# Autodesk Inventor assembly: tail
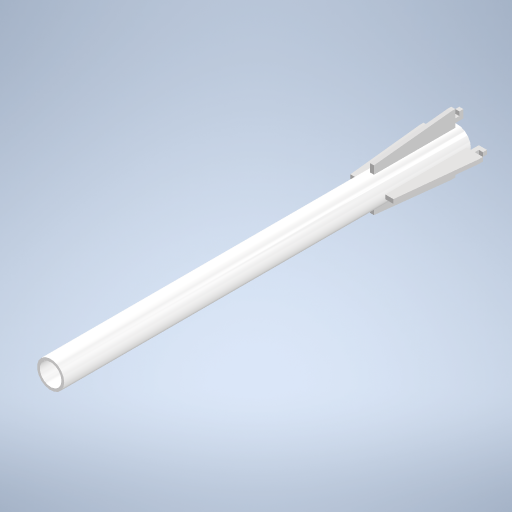
[picture p0: Inventor's stored thumbnail of the model, 512x512]
Saved by Autodesk Inventor 2023 (Build 270158000, 158)
## iProperties
Created: 2023-06-06
Part Number: tail
Document SubType Name: Assembly
Designer: Ronan
Author: Ronan
## Documents named in this file (3)
- D:\Libraries\Documents\2023-FYP\Inventor\tail.iam
- D:\Libraries\Documents\2023-FYP\Inventor\tail.ipt
- D:\Libraries\Documents\2023-FYP\Inventor\tail fin.ipt
## Components (5 placed, 2 different names)
1. tail:1 — Mate:1, Mate:2, Mate:3, Mate:4, Mate:5, Mate:6, Mate:7, Mate:8, Mate:9
2. tail fin:1 — Flush:1, Flush:2, Mate:4, Mate:5
3. tail fin:2 — Flush:1, Mate:6, Mate:7
4. tail fin:3 — Flush:2, Flush:3, Mate:1, Mate:2, Mate:3
5. tail fin:4 — Flush:3, Mate:8, Mate:9
## Relationships (12: Mate 9, Flush 3)
- Flush:1: tail fin:1 ↔ tail fin:2
- Flush:2: tail fin:1 ↔ tail fin:3
- Flush:3: tail fin:3 ↔ tail fin:4
- Mate:1: tail:1 ↔ tail fin:3
- Mate:2: tail:1 ↔ tail fin:3
- Mate:3: tail:1 ↔ tail fin:3
- Mate:4: tail:1 ↔ tail fin:1
- Mate:5: tail:1 ↔ tail fin:1
- Mate:6: tail:1 ↔ tail fin:2
- Mate:7: tail:1 ↔ tail fin:2
- Mate:8: tail:1 ↔ tail fin:4
- Mate:9: tail:1 ↔ tail fin:4
